# Autodesk Inventor assembly: Teleskopstange
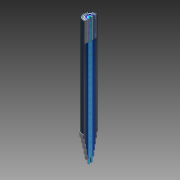
[picture p0: Inventor's stored thumbnail of the model, 180x180]
Saved by Autodesk Inventor 2012 SP1 (Build 160190100, 190)
## iProperties
Created: 2013-03-08
Part Number: Teleskopstange
Document SubType Name: Assembly
Designer: vogel
Author: vogel
## Documents named in this file (17)
- Z:\130204\Teleskopstange.iam
- Z:\130204\13_0204_022.ipt
- Z:\130204\13_0204_023.ipt
- Z:\130204\13_0204_024.ipt
- Z:\130204\13_0204_025.ipt
- Z:\130204\13_0204_026.ipt
- Z:\130204\13_0204_027.ipt
- Z:\130204\13_0204_030.ipt
- Z:\130204\13_0204_031.ipt
- Z:\130204\13_0204_032.ipt
- Z:\130204\13_0204_033.ipt
- Z:\130204\13_0204_035.ipt
- Z:\130204\13_0204_034.ipt
- Z:\130204\13_0204_036.ipt
- Z:\130204\13_0204_037.ipt
- Z:\130204\13_0204_038.ipt
- Z:\130204\13_0204_039.ipt
## Components (16 placed, 16 different names)
1. 13_0204_022:1 — Einfügen:64, Passend:95, A1
2. 13_0204_023:1 — Einfügen:49, Einfügen:51, A2, Passend:95, A1
3. 13_0204_024:1 — Einfügen:52, Passend:88, A3, Einfügen:66
4. 13_0204_025:1 — Einfügen:55, Passend:88, Einfügen:56, Passend:90, A4
5. 13_0204_026:1 — Einfügen:57, Passend:90, Einfügen:58, Passend:94, A5
6. 13_0204_027:1 — Einfügen:59, Passend:94
7. 13_0204_030:1 — Einfügen:49
8. 13_0204_031:1 — Einfügen:64
9. 13_0204_032:1 — Einfügen:52, A2
10. 13_0204_033:1 — Einfügen:51
11. 13_0204_035:1 — Einfügen:66
12. 13_0204_034:1 — Einfügen:55, A3
13. 13_0204_036:1 — Einfügen:57, A4
14. 13_0204_037:1 — Einfügen:56
15. 13_0204_038:1 — Einfügen:59, A5
16. 13_0204_039:1 — Einfügen:58
## Relationships (19: Insert 15, Mate 4)
- Einfügen:49 [Insert]: 13_0204_023:1 ↔ 13_0204_030:1
- Einfügen:51 [Insert]: 13_0204_023:1 ↔ 13_0204_033:1
- Einfügen:52 [Insert]: 13_0204_024:1 ↔ 13_0204_032:1
- A2 [Insert] (-237 mm): 13_0204_023:1 ↔ 13_0204_032:1
- Einfügen:55 [Insert]: 13_0204_025:1 ↔ 13_0204_034:1
- Passend:88 [Mate]: 13_0204_024:1 ↔ 13_0204_025:1
- Einfügen:56 [Insert]: 13_0204_025:1 ↔ 13_0204_037:1
- Einfügen:57 [Insert]: 13_0204_026:1 ↔ 13_0204_036:1
- Passend:90 [Mate]: 13_0204_025:1 ↔ 13_0204_026:1
- Einfügen:58 [Insert]: 13_0204_026:1 ↔ 13_0204_039:1
- Einfügen:59 [Insert]: 13_0204_027:1 ↔ 13_0204_038:1
- Passend:94 [Mate]: 13_0204_026:1 ↔ 13_0204_027:1
- A3 [Insert] (225 mm): 13_0204_024:1 ↔ 13_0204_034:1
- A4 [Insert] (-213 mm): 13_0204_025:1 ↔ 13_0204_036:1
- A5 [Insert] (-201 mm): 13_0204_026:1 ↔ 13_0204_038:1
- Einfügen:64 [Insert]: 13_0204_022:1 ↔ 13_0204_031:1
- Passend:95 [Mate]: 13_0204_022:1 ↔ 13_0204_023:1
- A1 [Insert]: 13_0204_022:1 ↔ 13_0204_023:1
- Einfügen:66 [Insert]: 13_0204_024:1 ↔ 13_0204_035:1
